# Autodesk Inventor assembly: osszeallitas
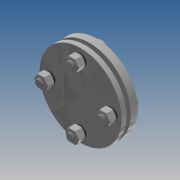
[picture p0: Inventor's stored thumbnail of the model, 180x180]
Saved by Autodesk Inventor 2016 (Build 200138000, 138)
## iProperties
Created: 2017-10-14
Part Number: osszeallitas
Document SubType Name: Assembly
Designer: Fauszt András V04MEA
Author: Fauszt András V04MEA
## Documents named in this file (7)
- C:\Users\Fauszt\Desktop\BME\Gép1\Model\osszeallitas.iam
- C:\Users\Fauszt\Desktop\BME\Gép1\Model\part.ipt
- C:\Users\Fauszt\Desktop\BME\Gép1\Model\vakkarima2.ipt
- C:\Users\Fauszt\Documents\Inventor\Content Center Files\R2016\en-US\ISO 8738(2)\ISO 8738 - 16(2).ipt
- C:\Users\Fauszt\Documents\Inventor\Content Center Files\R2016\en-US\ISO 4032(2)\ISO 4032 - M16 - ISO.ipt
- C:\Users\Fauszt\Desktop\BME\Gép1\Model\lapostomites2.ipt
- C:\Users\Fauszt\Documents\Inventor\Content Center Files\R2016\en-US\ISO 4017(1)\ISO 4017 - M16 x 55 - ISO.ipt
## Components (15 placed, 6 different names)
1. part:1 — Mate:5, Insert:1, Insert:2, Insert:3, Insert:4, Flush:2
2. vakkarima2:1 — Mate:4, Mate:5, Mate:7
3. lapostomites2:1 — Flush:2, Mate:4
4. ISO 4017 M16 x 55:1 — Insert:1, Mate:10
5. ISO 4017 M16 x 55:2 — Insert:2, Mate:14
6. ISO 4017 M16 x 55:3 — Insert:3, Mate:16
7. ISO 4017 M16 x 55:4 — Insert:4, Mate:12
8. ISO 4032 M16:5 — Mate:10, Mate:11
9. ISO 4032 M16:6 — Mate:12, Mate:13
10. ISO 4032 M16:7 — Mate:14, Mate:15
11. ISO 4032 M16:8 — Mate:16, Mate:17
12. ISO 8738 16:1 — Mate:7, Mate:11
13. ISO 8738 16:2 — Mate:13
14. ISO 8738 16:3 — Mate:15
15. ISO 8738 16:4 — Mate:17
## Component patterns: Alatet (4 elements)
## Relationships (16: Mate 11, Insert 4, Flush 1)
- Mate:4: vakkarima2:1 ↔ lapostomites2:1
- Mate:5: part:1 ↔ vakkarima2:1
- Mate:7: vakkarima2:1 ↔ ISO 8738 16:1
- Insert:1: part:1 ↔ ISO 4017 M16 x 55:1
- Insert:2: part:1 ↔ ISO 4017 M16 x 55:2
- Insert:3: part:1 ↔ ISO 4017 M16 x 55:3
- Insert:4: part:1 ↔ ISO 4017 M16 x 55:4
- Mate:10: ISO 4017 M16 x 55:1 ↔ ISO 4032 M16:5
- Mate:11: ISO 4032 M16:5 ↔ ISO 8738 16:1
- Mate:12: ISO 4017 M16 x 55:4 ↔ ISO 4032 M16:6
- Mate:13: ISO 4032 M16:6 ↔ ISO 8738 16:2
- Mate:14: ISO 4017 M16 x 55:2 ↔ ISO 4032 M16:7
- Mate:15: ISO 4032 M16:7 ↔ ISO 8738 16:3
- Mate:16: ISO 4017 M16 x 55:3 ↔ ISO 4032 M16:8
- Mate:17: ISO 4032 M16:8 ↔ ISO 8738 16:4
- Flush:2: part:1 ↔ lapostomites2:1
